# Autodesk Inventor assembly: ASY NDM-VOS_powder_hopper
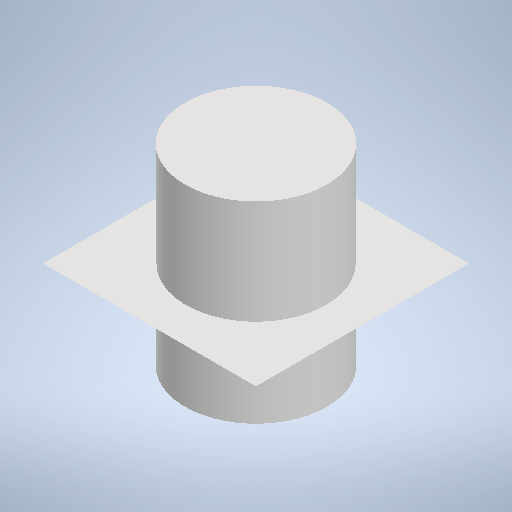
[picture p0: Inventor's stored thumbnail of the model, 512x512]
Saved by Autodesk Inventor 2025 (Build 290162010, 162A)
## iProperties
Created: 2024-07-24
Part Number: ASY NDM-VOS_powder_hopper
Document SubType Name: Assembly
Designer: admin
Author: admin
## Documents named in this file (4)
- C:\Users\user\YandexDisk\домашниий пк\Inventor\NDM-VOS_powder_hopper\ASY NDM-VOS_powder_hopper.iam
- C:\Users\user\YandexDisk\домашниий пк\Inventor\NDM-VOS_powder_hopper\NDM-VOS dummy1.ipt
- C:\Users\user\YandexDisk\домашниий пк\Inventor\NDM-VOS_powder_hopper\Dummy 3.ipt
- C:\Users\user\YandexDisk\домашниий пк\Inventor\NDM-VOS_powder_hopper\NDM-VOS dummy2.ipt
## Components (3 placed, 3 different names)
1. NDM-VOS dummy1:1
2. Dummy 3:1 — Flush:1
3. NDM-VOS dummy2:1 — Flush:2
## Relationships (2: Flush 2)
- Flush:1: Dummy 3:1
- Flush:2: NDM-VOS dummy2:1
